# Autodesk Inventor assembly: OktagonElektronik
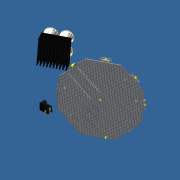
[picture p0: Inventor's stored thumbnail of the model, 180x180]
Saved by Autodesk Inventor 2018.2 (Build 222227000, 227)
## iProperties
Company: Fraunhofer ILT
Created: 2018-10-31
Part Number: OktagonElektronik
Material: geeigneten Werkstoff auswählen !
Document SubType Name: Assembly
Designer: N.Grubert
Title: =Description
Author: N.Grubert
## Documents named in this file (10)
- C:\Users\GRUBERT\Documents\COSIMA-Laserstar\CAD\Oktokommander\OktagonElektronik.iam
- C:\Users\GRUBERT\Documents\COSIMA-Laserstar\CAD\ARDUINO MICRO.iam
- C:\Users\GRUBERT\Documents\COSIMA-Laserstar\CAD\Polygonplatine.ipt
- C:\Users\GRUBERT\Documents\COSIMA-Laserstar\CAD\USB_female.ipt
- C:\Users\GRUBERT\Documents\COSIMA-Laserstar\CAD\Kühlkörper.ipt
- C:\Users\GRUBERT\Documents\COSIMA-Laserstar\CAD\Photodiodendummie.ipt
- C:\Users\GRUBERT\Documents\COSIMA-Laserstar\CAD\Parabol.ipt
- C:\Users\GRUBERT\Documents\COSIMA-Laserstar\CAD\16Bit I2C ADC+PGA - ADS1115.iam
- C:\Users\GRUBERT\Documents\COSIMA-Laserstar\CAD\Adafruit.ipt
- C:\Users\GRUBERT\Downloads\2-1mm-dc-power-socket\2.1mm_DC_Power_Socket.ipt
## Components (21 placed, 9 different names)
1. ARDUINO MICRO:1 [sub-assembly] — Fluchtend:1, Passend:18, Fluchtend:18
2. Polygonplatine:1 — Passend:1, Passend:2, Passend:3, Passend:4, Passend:5, Passend:6, Passend:7, Fluchtend:1, Winkel:4, Fluchtend:2, Fluchtend:3, Fluchtend:7, Fluchtend:8, Fluchtend:9, Fluchtend:10, Fluchtend:11, Fluchtend:12, Fluchtend:13, Winkel:5, Winkel:6, Passend:18, Fluchtend:18, Passend:19
3. USB_female:1 — Passend:2, Winkel:1, Fluchtend:5, Fluchtend:10
4. USB_female:2 — Passend:4, Winkel:4, Fluchtend:13
5. USB_female:3 — Passend:1, Winkel:2, Fluchtend:6, Fluchtend:7
6. USB_female:4 — Passend:3, Winkel:3, Fluchtend:3, Fluchtend:4
7. USB_female:5 — Passend:6, Winkel:3, Fluchtend:2, Fluchtend:4, Fluchtend:12
8. USB_female:6 — Passend:7, Winkel:2, Fluchtend:6, Fluchtend:8
9. USB_female:7 — Passend:5, Winkel:1, Fluchtend:5, Fluchtend:9, Fluchtend:11
10. Kühlkörper:1 — Winkel:5, Winkel:6, Passend:9, Passend:10, Passend:11, Passend:12, Winkel:7, Winkel:8, Passend:16, Passend:17
11. Photodiodendummie:1
12. Photodiodendummie:2
13. Photodiodendummie:3
14. Photodiodendummie:4
15. Parabol:1 — Passend:12, Fluchtend:14, Fluchtend:15, Passend:13, Fluchtend:16, Fluchtend:17
16. Parabol:2 — Passend:11, Fluchtend:14, Fluchtend:15, Passend:13, Passend:14
17. Parabol:3 — Passend:10, Fluchtend:16, Fluchtend:17, Passend:15, Winkel:7
18. Parabol:4 — Passend:9, Passend:14, Passend:15, Winkel:8, Passend:16, Passend:17
19. 16Bit I2C ADC+PGA - ADS1115:1 [sub-assembly]
20. Adafruit:1 — Passend:19
21. 2.1mm_DC_Power_Socket:1
## Relationships (44: Mate 18, Flush 18, Angle 8)
- Passend:1 [Mate]: Polygonplatine:1 ↔ USB_female:3
- Passend:2 [Mate]: Polygonplatine:1 ↔ USB_female:1
- Passend:3 [Mate]: Polygonplatine:1 ↔ USB_female:4
- Passend:4 [Mate]: Polygonplatine:1 ↔ USB_female:2
- Passend:5 [Mate]: Polygonplatine:1 ↔ USB_female:7
- Passend:6 [Mate]: Polygonplatine:1 ↔ USB_female:5
- Passend:7 [Mate]: Polygonplatine:1 ↔ USB_female:6
- Fluchtend:1 [Flush]: ARDUINO MICRO:1 ↔ Polygonplatine:1
- Winkel:1 [Angle] (180 deg): USB_female:1 ↔ USB_female:7
- Winkel:2 [Angle] (180 deg): USB_female:3 ↔ USB_female:6
- Winkel:3 [Angle] (180 deg): USB_female:4 ↔ USB_female:5
- Winkel:4 [Angle] (180 deg): Polygonplatine:1 ↔ USB_female:2
- Fluchtend:2 [Flush]: Polygonplatine:1 ↔ USB_female:5
- Fluchtend:3 [Flush]: Polygonplatine:1 ↔ USB_female:4
- Fluchtend:4 [Flush]: USB_female:4 ↔ USB_female:5
- Fluchtend:5 [Flush]: USB_female:1 ↔ USB_female:7
- Fluchtend:6 [Flush]: USB_female:3 ↔ USB_female:6
- Fluchtend:7 [Flush]: Polygonplatine:1 ↔ USB_female:3
- Fluchtend:8 [Flush]: Polygonplatine:1 ↔ USB_female:6
- Fluchtend:9 [Flush]: Polygonplatine:1 ↔ USB_female:7
- Fluchtend:10 [Flush]: Polygonplatine:1 ↔ USB_female:1
- Fluchtend:11 [Flush]: Polygonplatine:1 ↔ USB_female:7
- Fluchtend:12 [Flush]: Polygonplatine:1 ↔ USB_female:5
- Fluchtend:13 [Flush]: Polygonplatine:1 ↔ USB_female:2
- Winkel:5 [Angle] (0 deg): Polygonplatine:1 ↔ Kühlkörper:1
- Winkel:6 [Angle] (0 deg): Polygonplatine:1 ↔ Kühlkörper:1
- Passend:9 [Mate]: Kühlkörper:1 ↔ Parabol:4
- Passend:10 [Mate]: Kühlkörper:1 ↔ Parabol:3
- Passend:11 [Mate]: Kühlkörper:1 ↔ Parabol:2
- Passend:12 [Mate]: Kühlkörper:1 ↔ Parabol:1
- Fluchtend:14 [Flush]: Parabol:1 ↔ Parabol:2
- Fluchtend:15 [Flush]: Parabol:1 ↔ Parabol:2
- Passend:13 [Mate] (20 mm): Parabol:1 ↔ Parabol:2
- Fluchtend:16 [Flush]: Parabol:1 ↔ Parabol:3
- Fluchtend:17 [Flush] (20 mm): Parabol:1 ↔ Parabol:3
- Passend:14 [Mate] (20 mm): Parabol:2 ↔ Parabol:4
- Passend:15 [Mate] (20 mm): Parabol:3 ↔ Parabol:4
- Winkel:7 [Angle] (180 deg): Kühlkörper:1 ↔ Parabol:3
- Winkel:8 [Angle] (180 deg): Kühlkörper:1 ↔ Parabol:4
- Passend:16 [Mate] (9.1 mm): Kühlkörper:1 ↔ Parabol:4
- Passend:17 [Mate] (9.1 mm): Kühlkörper:1 ↔ Parabol:4
- Passend:18 [Mate]: ARDUINO MICRO:1 ↔ Polygonplatine:1
- Fluchtend:18 [Flush]: ARDUINO MICRO:1 ↔ Polygonplatine:1
- Passend:19 [Mate]: Polygonplatine:1 ↔ Adafruit:1
